# Autodesk Inventor assembly: handle_base
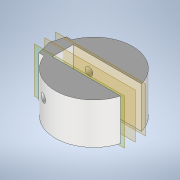
[picture p0: Inventor's stored thumbnail of the model, 180x180]
Saved by Autodesk Inventor 2022 (Build 260153000, 153)
## iProperties
Created: 2021-08-15
Part Number: handle_base
Document SubType Name: Assembly
Designer: teh18
Author: teh18
## Documents named in this file (3)
- C:\Users\ars-admin\Documents\GitHub\r68-bve-mascon\handle-base\handle_base.iam
- C:\Users\ars-admin\Documents\GitHub\r68-bve-mascon\handle-base\top.ipt
- C:\Users\ars-admin\Documents\GitHub\r68-bve-mascon\handle-base\bottom.ipt
## Components (2 placed, 2 different names)
1. top:1 — Mate:1, Angle:1, Mate:2, Angle:2
2. bottom:1
## Relationships (5: Mate 2, Angle 2, Symmetry 1)
- Mate:1: top:1
- Angle:1 (0 deg): top:1
- Mate:2: top:1
- Angle:2 (0 deg): top:1
- Symmetry:1
